# Autodesk Inventor assembly: PALM_asm
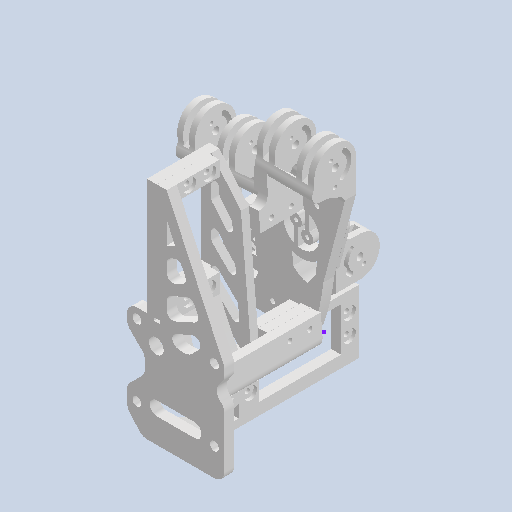
[picture p0: Inventor's stored thumbnail of the model, 512x512]
Saved by Autodesk Inventor 2025.2 (Build 292293000, 293)
## iProperties
Created: 2024-11-09
Part Number: PALM_asm
Document SubType Name: Assembly
Designer: esandor
Author: esandor
## Documents named in this file (5)
- C:\Users\esandor\Documents\Inventor\INDACT_EE\again\PALM\PALM_asm.iam
- C:\Users\esandor\Documents\Inventor\INDACT_EE\again\PALM\PALM_base.ipt
- C:\Users\esandor\Documents\Inventor\INDACT_EE\again\PALM\PALM_logo.ipt
- C:\Users\esandor\Documents\Inventor\INDACT_EE\again\PALM\PALM_lower_motor_holder.ipt
- C:\Users\esandor\Documents\Inventor\INDACT_EE\again\PALM\PALM_upper_motor_holder.ipt
## Components (4 placed, 4 different names)
1. PALM_base:1 — Mate:1, Insert:1, Insert:2, Mate:2, Insert:3, Insert:4, Mate:3, Insert:5, Insert:6
2. PALM_logo:1 — Mate:1, Insert:1, Insert:2
3. PALM_lower_motor_holder:1 — Mate:2, Insert:3, Insert:4
4. PALM_upper_motor_holder:1 — Mate:3, Insert:5, Insert:6
## Relationships (9: Insert 6, Mate 3)
- Mate:1: PALM_base:1 ↔ PALM_logo:1
- Insert:1: PALM_base:1 ↔ PALM_logo:1
- Insert:2: PALM_base:1 ↔ PALM_logo:1
- Mate:2: PALM_base:1 ↔ PALM_lower_motor_holder:1
- Insert:3: PALM_base:1 ↔ PALM_lower_motor_holder:1
- Insert:4: PALM_base:1 ↔ PALM_lower_motor_holder:1
- Mate:3: PALM_base:1 ↔ PALM_upper_motor_holder:1
- Insert:5: PALM_base:1 ↔ PALM_upper_motor_holder:1
- Insert:6: PALM_base:1 ↔ PALM_upper_motor_holder:1
